# Autodesk Inventor assembly: SG90 - Micro Servo 9g - Tower Pro
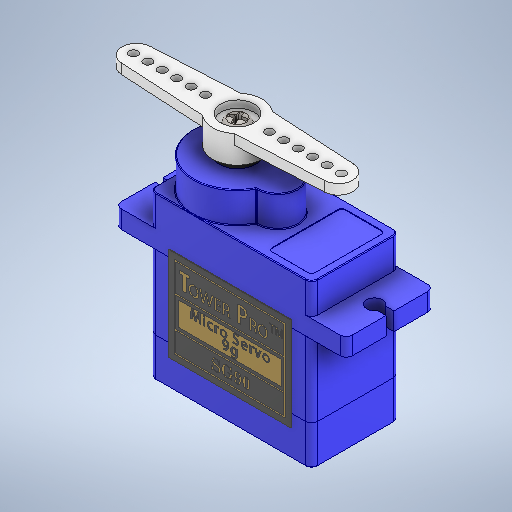
[picture p0: Inventor's stored thumbnail of the model, 512x512]
Saved by Autodesk Inventor 2027.1 (Build 311270010, 270A)
## iProperties
Created: 2019-03-11
Part Number: SG90 - Micro Servo 9g - Tower Pro
Description: STEP AP214
Document SubType Name: Assembly
Designer: chris
Sending System: SolidWorks 2018
Preprocessor: SwSTEP 2.0
Title: SG90 - Micro Servo 9g - Tower Pro.STEP
Revision Number: ANY
## Documents named in this file (4)
- C:\Users\chanh\Documents\RHp_Humanoid_ver1\Part_Body\Other Parts\head\SG90 - Micro Servo 9g - Tower Pro\SG90 - Micro Servo 9g - Tower Pro\SG90 - Micro Servo 9g - Tower Pro - bottom.iam
- C:\Users\chanh\Documents\RHp_Humanoid_ver1\Part_Body\Other Parts\head\SG90 - Micro Servo 9g - Tower Pro\SG90 - Micro Servo 9g - Tower Pro\SG90 - Micro Servo 9g - Tower Pro.1_Pea.ipt
- C:\Users\chanh\Documents\RHp_Humanoid_ver1\Part_Body\Other Parts\head\SG90 - Micro Servo 9g - Tower Pro\SG90 - Micro Servo 9g - Tower Pro\SG90 - Micro Servo 9g - Tower Pro.3_Pea.ipt
- C:\Users\chanh\Documents\RHp_Humanoid_ver1\Part_Body\Other Parts\head\SG90 - Micro Servo 9g - Tower Pro\SG90 - Micro Servo 9g - Tower Pro\SG90 - Micro Servo 9g - Tower Pro.6_BS EN ISO 7045 - M2 x 4 - Z - 4S.ipt
## Components (3 placed, 3 different names)
1. SG90 - Micro Servo 9g - Tower Pro.1_Pea_1 — Rotational:1
2. SG90 - Micro Servo 9g - Tower Pro.3_Pea_3 — Rotational:1, Rigid:1
3. SG90 - Micro Servo 9g - Tower Pro.6_BS EN ISO 7045 - M2 x 4 - Z - 4S_7 — Rigid:1
## Relationships (2: RevoluteJoint 1, WeldJoint 1)
- Rotational:1 [RevoluteJoint]: SG90 - Micro Servo 9g - Tower Pro.1_Pea_1 ↔ SG90 - Micro Servo 9g - Tower Pro.3_Pea_3
- Rigid:1 [WeldJoint]: SG90 - Micro Servo 9g - Tower Pro.3_Pea_3 ↔ SG90 - Micro Servo 9g - Tower Pro.6_BS EN ISO 7045 - M2 x 4 - Z - 4S_7
